# Autodesk Inventor assembly: RobotArm
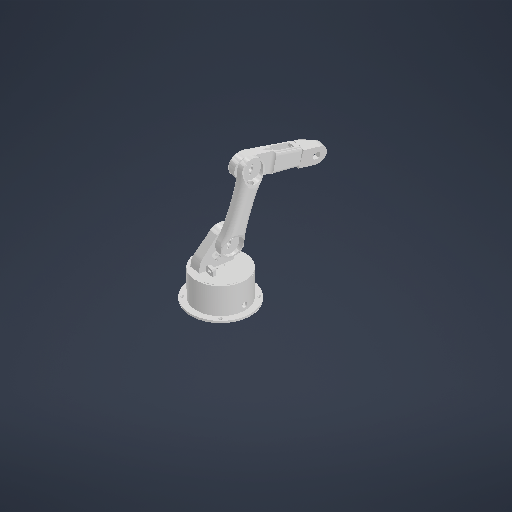
[picture p0: Inventor's stored thumbnail of the model, 512x512]
Saved by Autodesk Inventor 2025.1 (Build 291241000, 241)
## iProperties
Created: 2026-02-08
Part Number: RobotArm
Document SubType Name: Assembly
Designer: nikol
Author: nikol
## Documents named in this file (11)
- C:\Users\nikol\Documents\Inventor\TEK2602_SemPro\RobotArm.iam
- C:\Local\Nikolai\UIT\Y2\2_Semester\TEK-2602_Dronesystemer\sg90-micro-servo-9g-tower-pro-1.snapshot.3\SG90 - Micro Servo 9g - Tower Pro\Arm 01.ipt
- C:\Local\Nikolai\UIT\Y2\2_Semester\TEK-2602_Dronesystemer\sg90-micro-servo-9g-tower-pro-1.snapshot.3\SG90 - Micro Servo 9g - Tower Pro\Arm 02 v3.ipt
- C:\Local\Nikolai\UIT\Y2\2_Semester\TEK-2602_Dronesystemer\sg90-micro-servo-9g-tower-pro-1.snapshot.3\SG90 - Micro Servo 9g - Tower Pro\Arm 03.ipt
- C:\Local\Nikolai\UIT\Y2\2_Semester\TEK-2602_Dronesystemer\sg90-micro-servo-9g-tower-pro-1.snapshot.3\SG90 - Micro Servo 9g - Tower Pro\Base.ipt
- C:\Local\Nikolai\UIT\Y2\2_Semester\TEK-2602_Dronesystemer\sg90-micro-servo-9g-tower-pro-1.snapshot.3\SG90 - Micro Servo 9g - Tower Pro\gear1.ipt
- C:\Local\Nikolai\UIT\Y2\2_Semester\TEK-2602_Dronesystemer\sg90-micro-servo-9g-tower-pro-1.snapshot.3\SG90 - Micro Servo 9g - Tower Pro\gear2.ipt
- C:\Local\Nikolai\UIT\Y2\2_Semester\TEK-2602_Dronesystemer\sg90-micro-servo-9g-tower-pro-1.snapshot.3\SG90 - Micro Servo 9g - Tower Pro\grip link 1.ipt
- C:\Local\Nikolai\UIT\Y2\2_Semester\TEK-2602_Dronesystemer\sg90-micro-servo-9g-tower-pro-1.snapshot.3\SG90 - Micro Servo 9g - Tower Pro\Gripper 1.ipt
- C:\Local\Nikolai\UIT\Y2\2_Semester\TEK-2602_Dronesystemer\sg90-micro-servo-9g-tower-pro-1.snapshot.3\SG90 - Micro Servo 9g - Tower Pro\Gripper base.ipt
- C:\Local\Nikolai\UIT\Y2\2_Semester\TEK-2602_Dronesystemer\sg90-micro-servo-9g-tower-pro-1.snapshot.3\SG90 - Micro Servo 9g - Tower Pro\Waist.ipt
## Components (10 placed, 10 different names)
1. Arm 01:1 — Insert:2, Insert:3
2. Arm 02 v3:1 — Insert:3, Insert:4
3. Arm 03:1 — Insert:4
4. Base:1 — Insert:1
5. gear1:1
6. gear2:1
7. grip link 1:1
8. Gripper 1:1
9. Gripper base:1
10. Waist:1 — Insert:1, Insert:2
## Relationships (4: Insert 4)
- Insert:1: Base:1 ↔ Waist:1
- Insert:2: Arm 01:1 ↔ Waist:1
- Insert:3: Arm 01:1 ↔ Arm 02 v3:1
- Insert:4: Arm 02 v3:1 ↔ Arm 03:1
